# Autodesk Inventor assembly: preadator nano fixed mount template
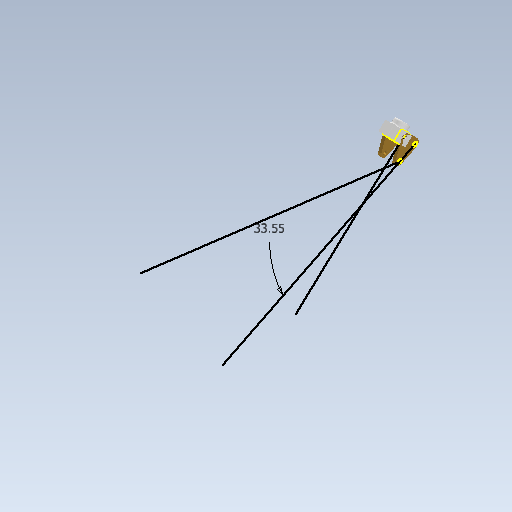
[picture p0: Inventor's stored thumbnail of the model, 512x512]
Saved by Autodesk Inventor 2020 (Build 240168000, 168)
## iProperties
Created: 2022-06-22
Part Number: preadator nano fixed mount template
Document SubType Name: Assembly
Designer: Steven
Author: Steven
## Documents named in this file (4)
- Y:\FPV drone stuff\0 Street League\Frames\PB-Kauri-X\3D prints\35 mm canopy\work in progress prints\Camera mounts\predator nano\preadator nano fixed mount template.iam
- Y:\FPV drone stuff\0 Street League\Frames\PB-Kauri-X\3D prints\35 mm canopy\Kauri modular camera mount HDzero micro v1 mirror.ipt
- Y:\FPV drone stuff\0 Street League\Frames\PB-Kauri-X\3D prints\35 mm canopy\Kauri modular camera mount HDzero micro v1.ipt
- Y:\FPV drone stuff\0 Street League\Frames\PB-Kauri-X\3D prints\35 mm canopy\work in progress prints\Camera mounts\predator nano\camera housing V1.ipt
## Components (3 placed, 3 different names)
1. Kauri modular camera mount HDzero micro v1 mirror:1 — Flush:1, Flush:2, Flush:3, Insert:1, Mate:1, Mate:3, Angle:1
2. Kauri modular camera mount HDzero micro v1:1 — Insert:1, Mate:1, Flush:4
3. camera housing V1:1 — Mate:3, Angle:1, Flush:4
## Relationships (8: Flush 4, Mate 2, Insert 1, Angle 1)
- Flush:1: Kauri modular camera mount HDzero micro v1 mirror:1
- Flush:2: Kauri modular camera mount HDzero micro v1 mirror:1
- Flush:3: Kauri modular camera mount HDzero micro v1 mirror:1
- Insert:1 (14.7 mm): Kauri modular camera mount HDzero micro v1 mirror:1 ↔ Kauri modular camera mount HDzero micro v1:1
- Mate:1: Kauri modular camera mount HDzero micro v1 mirror:1 ↔ Kauri modular camera mount HDzero micro v1:1
- Mate:3: Kauri modular camera mount HDzero micro v1 mirror:1 ↔ camera housing V1:1
- Angle:1 (-50 deg): Kauri modular camera mount HDzero micro v1 mirror:1 ↔ camera housing V1:1
- Flush:4: Kauri modular camera mount HDzero micro v1:1 ↔ camera housing V1:1
